# Autodesk Inventor assembly: lampu
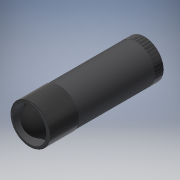
[picture p0: Inventor's stored thumbnail of the model, 180x180]
Saved by Autodesk Inventor 2019.5 (Build 235369000, 369)
## iProperties
Created: 2022-10-11
Part Number: lampu
Document SubType Name: Assembly
Designer: ASUS
Author: ASUS
## Documents named in this file (5)
- C:\Users\ASUS\Downloads\produk fri-074\lampu.iam
- C:\Users\ASUS\Downloads\produk fri-074\badan lampu.ipt
- C:\Users\ASUS\Downloads\produk fri-074\ttp lmp.iam
- C:\Users\ASUS\Downloads\produk fri-074\kaca lampu.ipt
- C:\Users\ASUS\Downloads\produk fri-074\kaca.ipt
## Components (4 placed, 4 different names)
1. badan lampu:2 — Mate:1, Mate:3
2. ttp lmp:1 [sub-assembly] — Mate:3
3. kaca lampu:1 — Mate:1, Mate:2
4. kaca:1 — Mate:2
## Relationships (3: Mate 3)
- Mate:1: badan lampu:2 ↔ kaca lampu:1
- Mate:2: kaca lampu:1 ↔ kaca:1
- Mate:3: badan lampu:2 ↔ ttp lmp:1
